# Autodesk Inventor assembly: Förderband
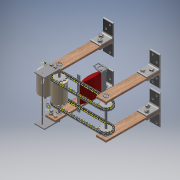
[picture p0: Inventor's stored thumbnail of the model, 180x180]
Saved by Autodesk Inventor 2018 (Build 220112000, 112)
## iProperties
Created: 2018-01-11
Part Number: Förderband
Material: Generisch
Document SubType Name: Assembly
Designer: Dominik
Author: Dominik
## Documents named in this file (17)
- C:\Users\Julian\Desktop\Schule\5AHME\Diplomarbeit\Git\fuettr_prototype\Mechanical\Inventorskizzen\Förderband.iam
- C:\Users\Julian\Desktop\Schule\5AHME\Diplomarbeit\Git\fuettr_prototype\Mechanical\Inventorskizzen\Kettenradzusammensetzung_links.iam
- C:\Users\Julian\Desktop\Schule\5AHME\Diplomarbeit\Git\fuettr_prototype\Mechanical\Inventorskizzen\Förderbandwelle_vorne.ipt
- C:\Users\Julian\Desktop\Schule\5AHME\Diplomarbeit\Git\fuettr_prototype\Mechanical\Inventorskizzen\Förderbandwelle_hinten.ipt
- C:\Users\Julian\Desktop\Schule\5AHME\Diplomarbeit\Git\fuettr_prototype\Mechanical\Inventorskizzen\Kunststoffrolle_antrieb.ipt
- C:\Users\Julian\Desktop\Schule\5AHME\Diplomarbeit\Git\fuettr_prototype\Mechanical\Inventorskizzen\Auspressrolle_befaesstigung.iam
- C:\Users\Julian\Documents\Inventor\Content Center Files\R2018\de-DE\DIN 471(1)\DIN 471 - 8x0,8.ipt
- C:\Users\Julian\Documents\Inventor\Content Center Files\R2018\de-DE\IS 2048  A\IS 2048 - 1983 - Spezifikation für Passfedern und Keilnute A 3 x 3 x 6.ipt
- C:\Users\Julian\Desktop\Schule\5AHME\Diplomarbeit\Git\fuettr_prototype\Mechanical\Inventorskizzen\Lagerhalterung.iam
- C:\Users\Julian\Desktop\Schule\5AHME\Diplomarbeit\Git\fuettr_prototype\Mechanical\Inventorskizzen\Lagerhalterung_ohne_Platte.iam
- C:\Users\Julian\Desktop\Schule\5AHME\Diplomarbeit\Git\fuettr_prototype\Mechanical\Inventorskizzen\Lagerhalterung_links.iam
- C:\Users\Julian\Desktop\Schule\5AHME\Diplomarbeit\Git\fuettr_prototype\Mechanical\Inventorskizzen\Bolzen_228.ipt
- C:\Users\Julian\Desktop\Schule\5AHME\Diplomarbeit\Git\fuettr_prototype\Mechanical\Inventorskizzen\Verbindungsstück_Rolle.ipt
- C:\Users\Julian\Desktop\Schule\5AHME\Diplomarbeit\Git\fuettr_prototype\Mechanical\Inventorskizzen\Platte_Kettenglied_unten.ipt
- C:\Users\Julian\Desktop\Schule\5AHME\Diplomarbeit\Git\fuettr_prototype\Mechanical\Inventorskizzen\Platte_Kettenglied_oben.ipt
- C:\Users\Julian\Desktop\Schule\5AHME\Diplomarbeit\Git\fuettr_prototype\Mechanical\Inventorskizzen\Futrterbeutel.ipt
- C:\Users\Julian\Desktop\Schule\5AHME\Diplomarbeit\Git\fuettr_prototype\Mechanical\Inventorskizzen\Hebel_Klemme.iam
## Components (29 placed, 16 different names)
1. Kettenradzusammensetzung_links:1 [sub-assembly] — Starr:2, Starr:5, Starr:6, Starr:15, Drehbar:21
2. Kettenradzusammensetzung_links:2 [sub-assembly] — Starr:1, Starr:4, Starr:13, Drehbar:22
3. Kunststoffrolle_antrieb:1 — Starr:3, Passend:1, Fluchtend:2
4. Förderbandwelle_hinten:1 — Starr:4, Starr:5, Starr:7, Starr:8, Starr:9, Starr:10, Starr:17, Starr:19
5. Förderbandwelle_vorne:1 — Starr:1, Starr:2, Starr:3, Drehbar:1, Starr:11, Starr:12, Starr:14, Starr:16, Drehbar:19, Fluchtend:1, Drehbar:2
6. Auspressrolle_befaesstigung:1 [sub-assembly] — Passend:1, Zylindrisch:1, Fluchtend:2, Zylindrisch:2, Passend:2, Passend:4, Passend:5, Passend:7
7. DIN 471 8x0,8:1 — Starr:7
8. DIN 471 8x0,8:2 — Starr:6
9. DIN 471 8x0,8:3 — Starr:13
10. DIN 471 8x0,8:5 — Starr:16
11. DIN 471 8x0,8:7 — Starr:15
12. DIN 471 8x0,8:9 — Starr:14
13. DIN 471 8x0,8:11 — Starr:12
14. DIN 471 8x0,8:12 — Starr:8
15. IS 2048 A Spezifikation für Passfedern und Keilnute A 3 x 3 x 6:1 — Drehbar:1
16. IS 2048 A Spezifikation für Passfedern und Keilnute A 3 x 3 x 6:2 — Starr:10
17. IS 2048 A Spezifikation für Passfedern und Keilnute A 3 x 3 x 6:3 — Starr:9
18. IS 2048 A Spezifikation für Passfedern und Keilnute A 3 x 3 x 6:4 — Starr:11
19. Lagerhalterung:2 [sub-assembly] — Drehbar:19, Fluchtend:1, Fluchtend:3, Zylindrisch:2, Drehbar:20
20. Lagerhalterung_ohne_Platte:1 [sub-assembly] — Starr:19
21. Lagerhalterung_ohne_Platte:2 [sub-assembly] — Starr:17
22. Lagerhalterung_links:1 [sub-assembly] — Drehbar:2, Zylindrisch:1, Fluchtend:3
23. Bolzen_228:1 — Drehbar:20, Passend:3, Passend:6
24. Verbindungsstück_Rolle:1 — Passend:2, Passend:3, Passend:4
25. Verbindungsstück_Rolle:2 — Passend:5, Passend:6, Passend:7
26. Platte_Kettenglied_unten:1 — Drehbar:21, Drehbar:22, Verschiebbar:1
27. Platte_Kettenglied_oben:1 — Starr:20
28. Futrterbeutel:1 — Verschiebbar:1, Starr:20, Starr:21
29. Hebel_Klemme:1 [sub-assembly] — Starr:21
## Relationships (39: WeldJoint 20, Mate 7, RevoluteJoint 6, Flush 3, CylindricalJoint 2, TranslationJoint 1)
- Starr:1 [WeldJoint]: Kettenradzusammensetzung_links:2 ↔ Förderbandwelle_vorne:1
- Starr:2 [WeldJoint]: Kettenradzusammensetzung_links:1 ↔ Förderbandwelle_vorne:1
- Starr:3 [WeldJoint]: Kunststoffrolle_antrieb:1 ↔ Förderbandwelle_vorne:1
- Starr:4 [WeldJoint]: Kettenradzusammensetzung_links:2 ↔ Förderbandwelle_hinten:1
- Starr:5 [WeldJoint]: Kettenradzusammensetzung_links:1 ↔ Förderbandwelle_hinten:1
- Starr:6 [WeldJoint]: Kettenradzusammensetzung_links:1 ↔ DIN 471 8x0,8:2
- Starr:7 [WeldJoint]: Förderbandwelle_hinten:1 ↔ DIN 471 8x0,8:1
- Starr:8 [WeldJoint]: Förderbandwelle_hinten:1 ↔ DIN 471 8x0,8:12
- Starr:9 [WeldJoint]: Förderbandwelle_hinten:1 ↔ IS 2048 A Spezifikation für Passfedern und Keilnute A 3 x 3 x 6:3
- Starr:10 [WeldJoint]: Förderbandwelle_hinten:1 ↔ IS 2048 A Spezifikation für Passfedern und Keilnute A 3 x 3 x 6:2
- Drehbar:1 [RevoluteJoint]: Förderbandwelle_vorne:1 ↔ IS 2048 A Spezifikation für Passfedern und Keilnute A 3 x 3 x 6:1
- Starr:11 [WeldJoint]: Förderbandwelle_vorne:1 ↔ IS 2048 A Spezifikation für Passfedern und Keilnute A 3 x 3 x 6:4
- Starr:12 [WeldJoint]: Förderbandwelle_vorne:1 ↔ DIN 471 8x0,8:11
- Starr:13 [WeldJoint]: Kettenradzusammensetzung_links:2 ↔ DIN 471 8x0,8:3
- Starr:14 [WeldJoint]: Förderbandwelle_vorne:1 ↔ DIN 471 8x0,8:9
- Starr:15 [WeldJoint]: Kettenradzusammensetzung_links:1 ↔ DIN 471 8x0,8:7
- Starr:16 [WeldJoint]: Förderbandwelle_vorne:1 ↔ DIN 471 8x0,8:5
- Passend:1 [Mate]: Kunststoffrolle_antrieb:1 ↔ Auspressrolle_befaesstigung:1
- Starr:17 [WeldJoint]: Förderbandwelle_hinten:1 ↔ Lagerhalterung_ohne_Platte:2
- Drehbar:19 [RevoluteJoint]: Förderbandwelle_vorne:1 ↔ Lagerhalterung:2
- Fluchtend:1 [Flush]: Förderbandwelle_vorne:1 ↔ Lagerhalterung:2
- Drehbar:2 [RevoluteJoint]: Förderbandwelle_vorne:1 ↔ Lagerhalterung_links:1
- Starr:19 [WeldJoint]: Förderbandwelle_hinten:1 ↔ Lagerhalterung_ohne_Platte:1
- Zylindrisch:1 [CylindricalJoint]: Auspressrolle_befaesstigung:1 ↔ Lagerhalterung_links:1
- Fluchtend:2 [Flush]: Kunststoffrolle_antrieb:1 ↔ Auspressrolle_befaesstigung:1
- Fluchtend:3 [Flush]: Lagerhalterung:2 ↔ Lagerhalterung_links:1
- Zylindrisch:2 [CylindricalJoint]: Auspressrolle_befaesstigung:1 ↔ Lagerhalterung:2
- Drehbar:20 [RevoluteJoint]: Lagerhalterung:2 ↔ Bolzen_228:1
- Passend:2 [Mate]: Auspressrolle_befaesstigung:1 ↔ Verbindungsstück_Rolle:1
- Passend:3 [Mate]: Bolzen_228:1 ↔ Verbindungsstück_Rolle:1
- Passend:4 [Mate]: Auspressrolle_befaesstigung:1 ↔ Verbindungsstück_Rolle:1
- Passend:5 [Mate]: Auspressrolle_befaesstigung:1 ↔ Verbindungsstück_Rolle:2
- Passend:6 [Mate]: Bolzen_228:1 ↔ Verbindungsstück_Rolle:2
- Passend:7 [Mate]: Auspressrolle_befaesstigung:1 ↔ Verbindungsstück_Rolle:2
- Drehbar:21 [RevoluteJoint]: Kettenradzusammensetzung_links:1 ↔ Platte_Kettenglied_unten:1
- Drehbar:22 [RevoluteJoint]: Kettenradzusammensetzung_links:2 ↔ Platte_Kettenglied_unten:1
- Verschiebbar:1 [TranslationJoint]: Platte_Kettenglied_unten:1 ↔ Futrterbeutel:1
- Starr:20 [WeldJoint]: Platte_Kettenglied_oben:1 ↔ Futrterbeutel:1
- Starr:21 [WeldJoint]: Futrterbeutel:1 ↔ Hebel_Klemme:1
